# Autodesk Inventor assembly: Z18936-S SHAFT ASSEMBLY
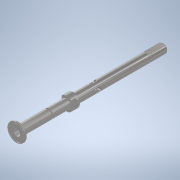
[picture p0: Inventor's stored thumbnail of the model, 180x180]
Saved by Autodesk Inventor 2021 (Build 250183000, 183)
## iProperties
Created: 2021-03-29
Part Number: Z18936-S SHAFT ASSEMBLY
Document SubType Name: Assembly
Designer: Work
Author: Work
Revision Number: 00
## Documents named in this file (3)
- C:\Users\Work\OneDrive - Brookhaven National Laboratory\Daniels, William intern HPR station\Arm\Z18936-S SHAFT ASSEMBLY.iam
- C:\Users\Work\OneDrive - Brookhaven National Laboratory\Daniels, William intern HPR station\Arm\Z18936-S1 SHAFT.ipt
- C:\Users\Work\OneDrive - Brookhaven National Laboratory\Daniels, William intern HPR station\Arm\Z18936-S2 BIOPHARM FITTING.ipt
## Components (2 placed, 2 different names)
1. Z18936-S1 SHAFT:1 — Rigid:1
2. Z18936-S2 BIOPHARM FITTING:1 — Rigid:1
## Relationships (1: WeldJoint 1)
- Rigid:1 [WeldJoint]: Z18936-S1 SHAFT:1 ↔ Z18936-S2 BIOPHARM FITTING:1
